# Autodesk Inventor assembly: Assembly
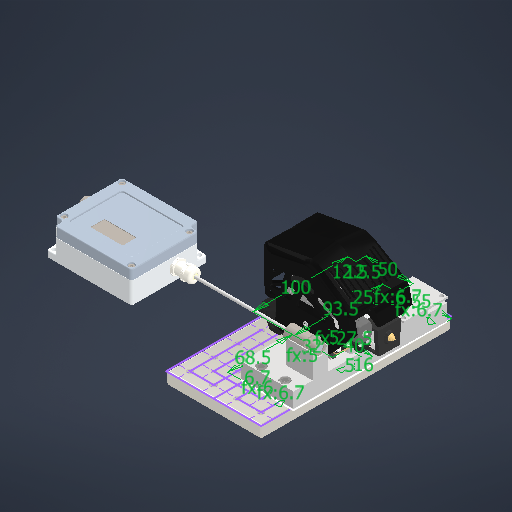
[picture p0: Inventor's stored thumbnail of the model, 512x512]
Saved by Autodesk Inventor 2027 (Build 310192060, 192F)
## iProperties
Created: 2026-07-09
Part Number: Assembly
Document SubType Name: Assembly
Designer: jacob
Author: jacob
## Documents named in this file (10)
- C:\Users\jacob\Documents\Autodesk\Inventor 2027\mount_proj_v3\Assembly.iam
- Mount_V1.1_Assembly.iam
- C:\Users\jacob\Documents\Autodesk\Inventor 2027\mount_proj_v3\Mount.ipt
- C:\Users\jacob\Documents\Autodesk\Inventor 2027\mount_proj_v3\sensors_printhead_mounts_consolidated.ipt
- C:\Users\jacob\OneDrive\Documents\Inventor\Content Center Files\R2027\en-US\ANSI B18.3.1M(6)\ANSI B18.3.1M - M6x1 x 12(1).ipt
- C:\Users\jacob\Documents\Autodesk\Inventor 2027\mount_proj_v3\M5 Bolt Derived.ipt
- C:\Users\jacob\Documents\Autodesk\Inventor 2027\mount_proj_v3\M5 Nut Derived.ipt
- C:\Users\jacob\Documents\Autodesk\Inventor 2027\mount_proj_v3\Ender_3_V3_SE_Derived.ipt
- C:\Users\jacob\Documents\Autodesk\Inventor 2027\mount_proj_v3\ILD1x20-500.ipt
- C:\Users\jacob\Documents\Autodesk\Inventor 2027\mount_proj_v3\thermoMETER UC.ipt
## Components (15 placed, 8 different names)
1. Mount:1 — Angle:2, Rotational:1, Angle:3, Angle:4
2. sensors_printhead_mounts_consolidated:1 — Rotational:1, Rotational:2, Rotational:3, Mate:1
3. Ender_3_V3_SE_Derived:1 — Angle:2
4. ILD1x20-500:1
5. thermoMETER UC:1 — Angle:3, Angle:4, Mate:1
6. M5_Nut_Derived:1
7. M5_Nut_Derived:2
8. M5_Nut_Derived:3
9. M5_Bolt_Derived:2
10. M5_Bolt_Derived:3
11. M5_Bolt_Derived:1
12. Forged Socket Head Cap Screw - Metric M6x1 x 12:1 — Rotational:3
13. Forged Socket Head Cap Screw - Metric M6x1 x 12:2
14. Forged Socket Head Cap Screw - Metric M6x1 x 12:3
15. Forged Socket Head Cap Screw - Metric M6x1 x 12:4 — Rotational:2
## Relationships (7: Angle 3, RevoluteJoint 3, Mate 1)
- Angle:2 (0 deg): Mount:1 ↔ Ender_3_V3_SE_Derived:1
- Rotational:1 [RevoluteJoint]: Mount:1 ↔ sensors_printhead_mounts_consolidated:1
- Rotational:2 [RevoluteJoint]: sensors_printhead_mounts_consolidated:1 ↔ Forged Socket Head Cap Screw - Metric M6x1 x 12:4
- Rotational:3 [RevoluteJoint]: sensors_printhead_mounts_consolidated:1 ↔ Forged Socket Head Cap Screw - Metric M6x1 x 12:1
- Angle:3 (0 deg): Mount:1 ↔ thermoMETER UC:1
- Angle:4 (0 deg): Mount:1 ↔ thermoMETER UC:1
- Mate:1: sensors_printhead_mounts_consolidated:1 ↔ thermoMETER UC:1
